# Autodesk Inventor assembly: birdeye_elbowUnit
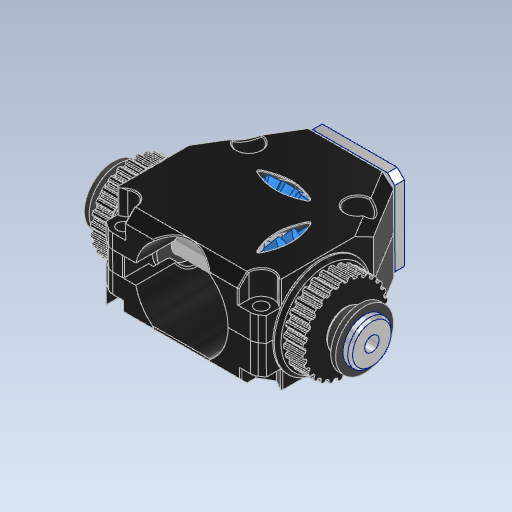
[picture p0: Inventor's stored thumbnail of the model, 512x512]
Saved by Autodesk Inventor 2024 (Build 280153000, 153)
## iProperties
Created: 2023-09-18
Part Number: birdeye_elbowUnit
Document SubType Name: Assembly
Designer: michi
Mass: 23.1104 g
Surface Area: 197.125 cm^2
Volume: 16.622 cm^3
Density: 1.39035 g/cm^3
Author: michi
## Documents named in this file (14)
- C:\Users\michi\OneDrive\default\robotis\DynamixelExamples\XC330MiniArm\birdeye_elbowUnit.iam
- C:\Users\michi\OneDrive\default\robotis\DynamixelExamples\XC330MiniArm\birdeye_elbowUnit\_GFM-0608-04.ipt
- C:\Users\michi\OneDrive\default\robotis\DynamixelExamples\XC330MiniArm\birdeye_elbowUnit\_SL-STWS6.ipt
- C:\Users\michi\OneDrive\default\robotis\DynamixelExamples\XC330MiniArm\birdeye_elbowUnit\brideye_elbowUnit_gearHolder_bottom.ipt
- C:\Users\michi\OneDrive\default\robotis\DynamixelExamples\XC330MiniArm\birdeye_elbowUnit\brideye_elbowUnit_pitchShaft.ipt
- C:\Users\michi\OneDrive\default\robotis\DynamixelExamples\XC330MiniArm\birdeye_elbowUnit\_B6701VV.ipt
- C:\Users\michi\OneDrive\default\robotis\DynamixelExamples\XC330MiniArm\birdeye_elbowUnit\brideye_elbowUnit_pully_passivePitch.ipt
- C:\Users\michi\OneDrive\default\robotis\DynamixelExamples\XC330MiniArm\birdeye_elbowUnit\brideye_elbowUnit_gearHolder_top.ipt
- C:\Users\michi\OneDrive\default\robotis\DynamixelExamples\XC330MiniArm\birdeye_elbowUnit\brideye_elbowUnit_pully_passiveRoll.ipt
- C:\Users\michi\OneDrive\default\robotis\DynamixelExamples\XC330MiniArm\birdeye_elbowUnit\_JFM-1214-05.ipt
- C:\Users\michi\OneDrive\default\robotis\DynamixelExamples\XC330MiniArm\birdeye_elbowUnit\brideye_elbowUnit_gear_active.ipt
- C:\Users\michi\OneDrive\default\robotis\DynamixelExamples\XC330MiniArm\birdeye_elbowUnit\brideye_elbowUnit_gear_passive.ipt
- C:\Users\michi\OneDrive\default\robotis\DynamixelExamples\XC330MiniArm\birdeye_elbowUnit\brideye_elbowUnit_rollShaft.ipt
- C:\Users\michi\OneDrive\default\robotis\DynamixelExamples\XC330MiniArm\birdeye_elbowUnit\brideye_elbowUnit_rollShaftConn.ipt
## Components (17 placed, 13 different names)
1. brideye_elbowUnit_gearHolder_bottom:1 — メイト:1, メイト:2, メイト:14, メイト:29, メイト:30, メイト:31, メイト:32, メイト:34
2. brideye_elbowUnit_gearHolder_top:1 — メイト:32, メイト:33, メイト:34, 角度:1
3. _GFM-0608-04:1 — メイト:18, メイト:19, メイト:20
4. _GFM-0608-04:2 — メイト:4, メイト:5, メイト:7
5. _GFM-0608-04:3 — メイト:3, メイト:6, メイト:20
6. _GFM-0608-04:4 — メイト:17, メイト:21, メイト:22
7. _SL-STWS6:1 — メイト:15, メイト:16, メイト:19
8. brideye_elbowUnit_pitchShaft:1 — メイト:7, メイト:9, メイト:10, メイト:15, メイト:16, メイト:17, メイト:18, メイト:21
9. _B6701VV:1 — メイト:23, メイト:27, メイト:31
10. _B6701VV:2 — メイト:24, メイト:25, メイト:28, メイト:29, メイト:30
11. brideye_elbowUnit_pully_passivePitch:1 — メイト:1, メイト:2, メイト:3, メイト:4, メイト:5, メイト:6, メイト:33
12. brideye_elbowUnit_pully_passiveRoll:1 — メイト:8, メイト:10, メイト:12, メイト:22
13. _JFM-1214-05:1 — メイト:11, メイト:12, メイト:13, メイト:14
14. brideye_elbowUnit_gear_active:1 — メイト:8, メイト:9, メイト:11, メイト:13
15. brideye_elbowUnit_gear_passive:1 — メイト:23, メイト:24, メイト:26, メイト:27, 回転:1
16. brideye_elbowUnit_rollShaft:1 — メイト:25, メイト:26, メイト:28, 角度:1
17. brideye_elbowUnit_rollShaftConn:1 — 回転:1
## Relationships (36: Mate 34, RevoluteJoint 1, Angle 1)
- メイト:1 [Mate]: brideye_elbowUnit_gearHolder_bottom:1 ↔ brideye_elbowUnit_pully_passivePitch:1
- メイト:2 [Mate]: brideye_elbowUnit_gearHolder_bottom:1 ↔ brideye_elbowUnit_pully_passivePitch:1
- メイト:3 [Mate]: _GFM-0608-04:3 ↔ brideye_elbowUnit_pully_passivePitch:1
- メイト:4 [Mate]: _GFM-0608-04:2 ↔ brideye_elbowUnit_pully_passivePitch:1
- メイト:5 [Mate]: _GFM-0608-04:2 ↔ brideye_elbowUnit_pully_passivePitch:1
- メイト:6 [Mate]: _GFM-0608-04:3 ↔ brideye_elbowUnit_pully_passivePitch:1
- メイト:7 [Mate]: _GFM-0608-04:2 ↔ brideye_elbowUnit_pitchShaft:1
- メイト:8 [Mate]: brideye_elbowUnit_pully_passiveRoll:1 ↔ brideye_elbowUnit_gear_active:1
- メイト:9 [Mate]: brideye_elbowUnit_pitchShaft:1 ↔ brideye_elbowUnit_gear_active:1
- メイト:10 [Mate]: brideye_elbowUnit_pitchShaft:1 ↔ brideye_elbowUnit_pully_passiveRoll:1
- メイト:11 [Mate]: _JFM-1214-05:1 ↔ brideye_elbowUnit_gear_active:1
- メイト:12 [Mate]: brideye_elbowUnit_pully_passiveRoll:1 ↔ _JFM-1214-05:1
- メイト:13 [Mate]: _JFM-1214-05:1 ↔ brideye_elbowUnit_gear_active:1
- メイト:14 [Mate]: brideye_elbowUnit_gearHolder_bottom:1 ↔ _JFM-1214-05:1
- メイト:15 [Mate]: _SL-STWS6:1 ↔ brideye_elbowUnit_pitchShaft:1
- メイト:16 [Mate]: _SL-STWS6:1 ↔ brideye_elbowUnit_pitchShaft:1
- メイト:17 [Mate]: _GFM-0608-04:4 ↔ brideye_elbowUnit_pitchShaft:1
- メイト:18 [Mate]: _GFM-0608-04:1 ↔ brideye_elbowUnit_pitchShaft:1
- メイト:19 [Mate]: _GFM-0608-04:1 ↔ _SL-STWS6:1
- メイト:20 [Mate]: _GFM-0608-04:1 ↔ _GFM-0608-04:3
- メイト:21 [Mate]: _GFM-0608-04:4 ↔ brideye_elbowUnit_pitchShaft:1
- メイト:22 [Mate]: _GFM-0608-04:4 ↔ brideye_elbowUnit_pully_passiveRoll:1
- メイト:23 [Mate]: _B6701VV:1 ↔ brideye_elbowUnit_gear_passive:1
- メイト:24 [Mate]: _B6701VV:2 ↔ brideye_elbowUnit_gear_passive:1
- メイト:25 [Mate]: _B6701VV:2 ↔ brideye_elbowUnit_rollShaft:1
- メイト:26 [Mate]: brideye_elbowUnit_gear_passive:1 ↔ brideye_elbowUnit_rollShaft:1
- メイト:27 [Mate]: _B6701VV:1 ↔ brideye_elbowUnit_gear_passive:1
- メイト:28 [Mate]: _B6701VV:2 ↔ brideye_elbowUnit_rollShaft:1
- メイト:29 [Mate]: brideye_elbowUnit_gearHolder_bottom:1 ↔ _B6701VV:2
- メイト:30 [Mate]: brideye_elbowUnit_gearHolder_bottom:1 ↔ _B6701VV:2
- メイト:31 [Mate]: brideye_elbowUnit_gearHolder_bottom:1 ↔ _B6701VV:1
- メイト:32 [Mate]: brideye_elbowUnit_gearHolder_bottom:1 ↔ brideye_elbowUnit_gearHolder_top:1
- メイト:33 [Mate]: brideye_elbowUnit_gearHolder_top:1 ↔ brideye_elbowUnit_pully_passivePitch:1
- メイト:34 [Mate]: brideye_elbowUnit_gearHolder_bottom:1 ↔ brideye_elbowUnit_gearHolder_top:1
- 回転:1 [RevoluteJoint]: brideye_elbowUnit_gear_passive:1 ↔ brideye_elbowUnit_rollShaftConn:1
- 角度:1 [Angle] (0 deg): brideye_elbowUnit_gearHolder_top:1 ↔ brideye_elbowUnit_rollShaft:1
